# Autodesk Inventor assembly: 3_CIM_Ball_Shifter_Base_Kit_with_3rd_Stage_217-3268_MIR
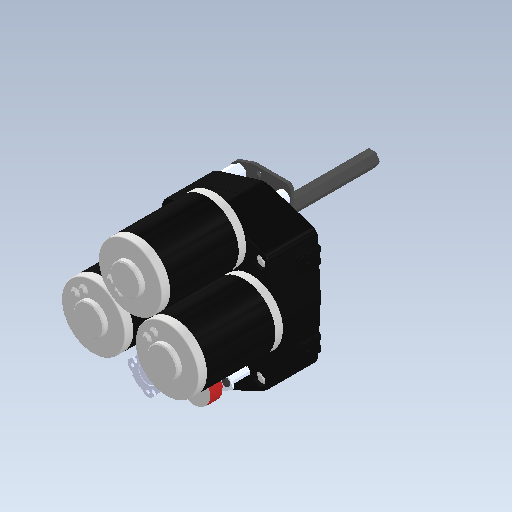
[picture p0: Inventor's stored thumbnail of the model, 512x512]
Saved by Autodesk Inventor 2020 (Build 240168000, 168)
## iProperties
Created: 2015-12-17
Part Number: 3_CIM_Ball_Shifter_Base_Kit_with_3rd_Stage_217-3268_MIR
Description: STEP AP214
Document SubType Name: Assembly
Designer: srini
Title: 217-3268-STEP-20151217.STEP
Revision Number: ANY
Sending System: SolidWorks 2015
Preprocessor: SwSTEP 2.0
## Documents named in this file (56)
- C:\Users\srini\Documents\FRC\2020\SuperShifter\3_CIM_Ball_Shifter_Base_Kit_with_3rd_Stage_217-3268_MIR.iam
- C:\Users\srini\Documents\FRC\2020\SuperShifter\217-2733-001 Rev2_MIR.ipt
- C:\Users\srini\Documents\FRC\2020\SuperShifter\217-2731-001 Rev2_MIR.ipt
- C:\Users\srini\Documents\FRC\2020\SuperShifter\217-2789-001 Rev2_MIR.ipt
- C:\Users\srini\Documents\FRC\2020\SuperShifter\217-2778-001 Rev2_NCQ8A075-050M_MIR.iam
- C:\Users\srini\Documents\FRC\2020\SuperShifter\217-2428-012 Rev2_MIR.ipt
- C:\Users\srini\Documents\FRC\2020\SuperShifter\217-2428-005 Rev1_MIR.ipt
- C:\Users\srini\Documents\FRC\2020\SuperShifter\SCREW-832-0375_MIR.ipt
- C:\Users\srini\Documents\FRC\2020\SuperShifter\SBS1_SBS-0632-0250_MIR.ipt
- C:\Users\srini\Documents\FRC\2020\SuperShifter\217-4098-100 Rev1_MIR.iam
- C:\Users\srini\Documents\FRC\2020\SuperShifter\217-2428-017 Rev2_MIR.ipt
- C:\Users\srini\Documents\FRC\2020\SuperShifter\217-2428-016 Rev3_Spur01_MIR.ipt
- C:\Users\srini\Documents\FRC\2020\SuperShifter\217-2428-019 Rev1_MIR.ipt
- C:\Users\srini\Documents\FRC\2020\SuperShifter\217-2428-006 Rev1_MIR.ipt
- C:\Users\srini\Documents\FRC\2020\SuperShifter\217-2614-001_12t_MIR.ipt
- C:\Users\srini\Documents\FRC\2020\SuperShifter\217-2761-001 rev1_MIR.ipt
- C:\Users\srini\Documents\FRC\2020\SuperShifter\217-3195-002 rev2_MIR.ipt
- C:\Users\srini\Documents\FRC\2020\SuperShifter\217-3195-001 Rev1_MIR.ipt
- C:\Users\srini\Documents\FRC\2020\SuperShifter\276-1027-001_MIR.ipt
- C:\Users\srini\Documents\FRC\2020\SuperShifter\SCREW-832-1750_MIR.ipt
- C:\Users\srini\Documents\FRC\2020\SuperShifter\217-2428-004 Rev3_MIR.ipt
- C:\Users\srini\Documents\FRC\2020\SuperShifter\217-2428-021 Rev1_MIR.ipt
- C:\Users\srini\Documents\FRC\2020\SuperShifter\217-2428-029 Rev1_MIR.ipt
- C:\Users\srini\Documents\FRC\2020\SuperShifter\Grayhill Lock Washer_MIR.ipt
- C:\Users\srini\Documents\FRC\2020\SuperShifter\Grayhill Nut_MIR.ipt
- C:\Users\srini\Documents\FRC\2020\SuperShifter\Grahill Encoder_MIR.ipt
- C:\Users\srini\Documents\FRC\2020\SuperShifter\SBS1_SBS-2520-125_MIR.ipt
- C:\Users\srini\Documents\FRC\2020\SuperShifter\217-3195-008 Rev1_stubby .75__MIR.ipt
- C:\Users\srini\Documents\FRC\2020\SuperShifter\Nylock Nut_NNY2520-ZC_MIR.ipt
- C:\Users\srini\Documents\FRC\2020\SuperShifter\SBS1_SBS2520-0625ZC_MIR.ipt
- C:\Users\srini\Documents\FRC\2020\SuperShifter\217-2617-002 Rev1_91780A359_MIR.ipt
- C:\Users\srini\Documents\FRC\2020\SuperShifter\217-3195-003 rev2_MIR.ipt
- C:\Users\srini\Documents\FRC\2020\SuperShifter\217-2617-003 Rev1_MIR.ipt
- C:\Users\srini\Documents\FRC\2020\SuperShifter\217-3109-001 Rev1_MIR.ipt
- C:\Users\srini\Documents\FRC\2020\SuperShifter\217-2734-001 Rev3_MIR.ipt
- C:\Users\srini\Documents\FRC\2020\SuperShifter\217-2617-004 Rev1_97431A340_grv_MIR.ipt
- C:\Users\srini\Documents\FRC\2020\SuperShifter\217-2702-001_20t_MIR.ipt
- C:\Users\srini\Documents\FRC\2020\SuperShifter\217-2715-002 Rev1_64t_MIR.ipt
- C:\Users\srini\Documents\FRC\2020\SuperShifter\217-2704-001_24_MIR.ipt
- C:\Users\srini\Documents\FRC\2020\SuperShifter\217-2714-002 Rev1_60t_MIR.ipt
- C:\Users\srini\Documents\FRC\2020\SuperShifter\217-3221-002 Rev1_MIR.ipt
- C:\Users\srini\Documents\FRC\2020\SuperShifter\217-2705-001_30t_MIR.ipt
- C:\Users\srini\Documents\FRC\2020\SuperShifter\217-2712-002 Rev1_50t_MIR.ipt
- C:\Users\srini\Documents\FRC\2020\SuperShifter\217-2706-001_34t_MIR.ipt
- C:\Users\srini\Documents\FRC\2020\SuperShifter\217-3287-001 Rev3_MIR.iam
- C:\Users\srini\Documents\FRC\2020\SuperShifter\217-3211-001 Rev1_34t_MIR.ipt
- C:\Users\srini\Documents\FRC\2020\SuperShifter\217-3288-001 Rev3_MIR.iam
- C:\Users\srini\Documents\FRC\2020\SuperShifter\217-3210-001 Rev1_30t_MIR.ipt
- C:\Users\srini\Documents\FRC\2020\SuperShifter\217-3292-001 Rev3_MIR.iam
- C:\Users\srini\Documents\FRC\2020\SuperShifter\217-2703-001_MIR.ipt
- C:\Users\srini\Documents\FRC\2020\SuperShifter\217-2711-002 Rev1_50t_MIR.ipt
- C:\Users\srini\Documents\FRC\2020\SuperShifter\217-2428-023 Rev1_9714K3_MIR.ipt
- C:\Users\srini\Documents\FRC\2020\SuperShifter\SBS_SBS2520-1750_MIR.ipt
- C:\Users\srini\Documents\FRC\2020\SuperShifter\NNYXXXX-ZZ_NNY2520-ZC_MIR.ipt
- C:\Users\srini\Documents\FRC\2020\SuperShifter\SBS_SBS2520-1500ZC_MIR.ipt
- C:\Users\srini\Documents\FRC\2020\SuperShifter\Mini_CIM_Motor_217-3371_MIR.ipt
## Components (83 placed, 55 different names)
1. 217-2733-001 Rev2_MIR:1
2. 217-2733-001 Rev2_MIR:2
3. 217-2731-001 Rev2_MIR:1
4. 217-2789-001 Rev2_MIR:1
5. 217-2778-001 Rev2_NCQ8A075-050M_MIR:1 [sub-assembly]
6. 217-2428-012 Rev2_MIR:1
7. 217-2428-005 Rev1_MIR:1
8. 217-2428-005 Rev1_MIR:2
9. SCREW-832-0375_MIR:1
10. SCREW-832-0375_MIR:2
11. SCREW-832-0375_MIR:3
12. SCREW-832-0375_MIR:4
13. SBS1_SBS-0632-0250_MIR:1
14. SBS1_SBS-0632-0250_MIR:2
15. 217-4098-100 Rev1_MIR:1 [sub-assembly]
16. 217-2428-017 Rev2_MIR:1
17. 217-2428-016 Rev3_Spur01_MIR:1
18. 217-2428-019 Rev1_MIR:1
19. 217-2428-006 Rev1_MIR:1
20. 217-2428-006 Rev1_MIR:2
21. SCREW-832-0375_MIR:5
22. SCREW-832-0375_MIR:6
23. SCREW-832-0375_MIR:7
24. SCREW-832-0375_MIR:8
25. 217-2614-001_12t_MIR:1
26. 217-2761-001 rev1_MIR:1
27. 217-2761-001 rev1_MIR:2
28. 217-2614-001_12t_MIR:2
29. 217-2614-001_12t_MIR:3
30. 217-2761-001 rev1_MIR:3
31. 217-3195-002 rev2_MIR:1
32. 217-3195-001 Rev1_MIR:1 — Insert:4, Insert:3, Insert:2, Insert:1, Insert:6, Insert:5
33. 276-1027-001_MIR:1
34. 276-1027-001_MIR:2
35. SCREW-832-1750_MIR:1
36. SCREW-832-1750_MIR:2
37. 217-2428-004 Rev3_MIR:1
38. 217-2428-021 Rev1_MIR:1
39. 217-2428-029 Rev1_MIR:1
40. Grayhill Lock Washer_MIR:1
41. Grayhill Nut_MIR:1
42. Grahill Encoder_MIR:1
43. SBS1_SBS-2520-125_MIR:1
44. 217-3195-008 Rev1_stubby .75__MIR:1
45. 217-3195-008 Rev1_stubby .75__MIR:2
46. Nylock Nut_NNY2520-ZC_MIR:1
47. Nylock Nut_NNY2520-ZC_MIR:2
48. SBS1_SBS2520-0625ZC_MIR:1
49. SBS1_SBS2520-0625ZC_MIR:2
50. 217-2617-002 Rev1_91780A359_MIR:1
51. 217-2617-002 Rev1_91780A359_MIR:2
52. 217-3195-003 rev2_MIR:1
53. 217-2617-003 Rev1_MIR:1
54. 217-3109-001 Rev1_MIR:1
55. 217-2734-001 Rev3_MIR:1
56. 217-2617-004 Rev1_97431A340_grv_MIR:1
57. 217-2617-004 Rev1_97431A340_grv_MIR:2
58. 217-2702-001_20t_MIR:1
59. 217-2715-002 Rev1_64t_MIR:1
60. 217-2704-001_24_MIR:1
61. 217-2714-002 Rev1_60t_MIR:1
62. 217-3221-002 Rev1_MIR:1
63. 217-2705-001_30t_MIR:1
64. 217-2712-002 Rev1_50t_MIR:1
65. 217-2706-001_34t_MIR:1
66. SBS1_SBS-2520-125_MIR:2
67. 217-3287-001 Rev3_MIR:1 [sub-assembly]
68. 217-3211-001 Rev1_34t_MIR:1
69. 217-3288-001 Rev3_MIR:1 [sub-assembly]
70. 217-3210-001 Rev1_30t_MIR:1
71. 217-3292-001 Rev3_MIR:1 [sub-assembly]
72. 217-2703-001_MIR:1
73. 217-2711-002 Rev1_50t_MIR:1
74. 217-2428-023 Rev1_9714K3_MIR:1
75. SBS_SBS2520-1750_MIR:1
76. SBS_SBS2520-1750_MIR:2
77. NNYXXXX-ZZ_NNY2520-ZC_MIR:1
78. NNYXXXX-ZZ_NNY2520-ZC_MIR:2
79. SBS_SBS2520-1500ZC_MIR:1
80. SBS_SBS2520-1500ZC_MIR:2
81. Mini_CIM_Motor_217-3371_MIR:1 — Insert:4, Insert:3
82. Mini_CIM_Motor_217-3371_MIR:2 — Insert:2, Insert:1
83. Mini_CIM_Motor_217-3371_MIR:3 — Insert:6, Insert:5
## Relationships (6: Insert 6)
- Insert:4: 217-3195-001 Rev1_MIR:1 ↔ Mini_CIM_Motor_217-3371_MIR:1
- Insert:3: 217-3195-001 Rev1_MIR:1 ↔ Mini_CIM_Motor_217-3371_MIR:1
- Insert:2: 217-3195-001 Rev1_MIR:1 ↔ Mini_CIM_Motor_217-3371_MIR:2
- Insert:1: 217-3195-001 Rev1_MIR:1 ↔ Mini_CIM_Motor_217-3371_MIR:2
- Insert:6: 217-3195-001 Rev1_MIR:1 ↔ Mini_CIM_Motor_217-3371_MIR:3
- Insert:5: 217-3195-001 Rev1_MIR:1 ↔ Mini_CIM_Motor_217-3371_MIR:3
